# Autodesk Inventor assembly: Assembly1
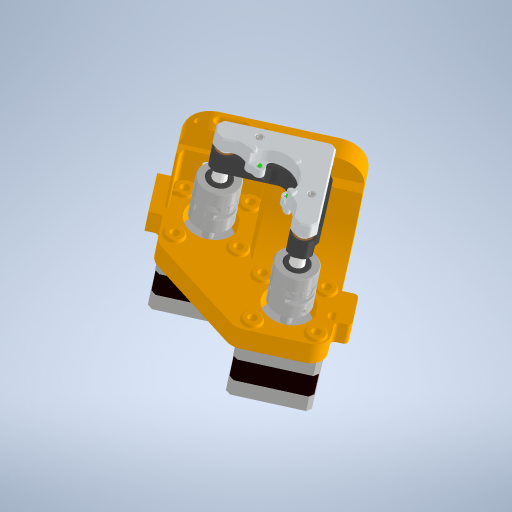
[picture p0: Inventor's stored thumbnail of the model, 512x512]
Saved by Autodesk Inventor 2024 (Build 280153000, 153)
## iProperties
Created: 2022-02-09
Part Number: Assembly1
Document SubType Name: Assembly
Designer: la8011
Author: la8011
## Documents named in this file (7)
- C:\Users\Mohamed Shehata\Dropbox (Dropbox @RU)\Design_mirror_control\Parts_assembly_final_GH\Motor_mirror_mount.iam
- C:\Users\Mohamed Shehata\Dropbox (Dropbox @RU)\Design_mirror_control\Parts_assembly_final_GH\Parts\KM1CE-Step.ipt
- C:\Users\Mohamed Shehata\Dropbox (Dropbox @RU)\Design_mirror_control\Parts_assembly_final_GH\Parts\Stage.ipt
- C:\Users\Mohamed Shehata\Dropbox (Dropbox @RU)\Design_mirror_control\Parts_assembly_final_GH\Parts\stepper.ipt
- C:\Users\Mohamed Shehata\Dropbox (Dropbox @RU)\Scan_DMD\Parts\59985K14_High-Parallel-Misalignment Flexible Shaft Coupling\59985K14_High-Parallel-Misalignment Flexible Shaft Coupling.ipt
- C:\Users\Mohamed Shehata\Dropbox (Dropbox @RU)\Scan_DMD\Parts\59985K62_93 in.-lbs. Acetal Disc for 3 4 OD High-Parallel-Misalignment Flexible Shaft Coupling\59985K62_93 in.-lbs. Acetal Disc for 3 4 OD High-Para.ipt
- C:\Users\Mohamed Shehata\Dropbox (Dropbox @RU)\Scan_DMD\Parts\59985K202_High-Parallel-Misalignment Flexible Shaft Coupling\59985K202_High-Parallel-Misalignment Flexible Shaft Coupling.ipt
## Components (10 placed, 6 different names)
1. KM1CE-Step:1 — Insert:1, Angle:3, Mate:7, Mate:14, Mate:15
2. Stage:1 — Insert:1, Angle:1, Angle:2, Angle:3, Mate:8, Mate:10, Mate:11
3. stepper:1 — Angle:1, Mate:7, Mate:8, Mate:13, Angle:6, Angle:7
4. stepper:2 — Angle:2, Mate:10, Mate:11, Mate:12, Angle:4, Angle:5
5. 59985K14_High-Parallel-Misalignment Flexible Shaft Coupling:1 — Angle:7, Mate:15, Mate:20, Mate:23
6. 59985K62_93 in.-lbs. Acetal Disc for 3 4 OD High-Para:1 — Mate:20, Mate:21, Mate:22, Mate:23
7. 59985K202_High-Parallel-Misalignment Flexible Shaft Coupling:1 — Mate:13, Angle:6, Mate:21, Mate:22
8. 59985K14_High-Parallel-Misalignment Flexible Shaft Coupling:2 — Mate:14, Angle:5, Mate:17, Mate:19
9. 59985K62_93 in.-lbs. Acetal Disc for 3 4 OD High-Para:2 — Mate:16, Mate:17, Mate:18, Mate:19
10. 59985K202_High-Parallel-Misalignment Flexible Shaft Coupling:2 — Mate:12, Angle:4, Mate:16, Mate:18
## Relationships (24: Mate 16, Angle 7, Insert 1)
- Insert:1: KM1CE-Step:1 ↔ Stage:1
- Angle:1 (0 deg): Stage:1 ↔ stepper:1
- Angle:2 (0 deg): Stage:1 ↔ stepper:2
- Angle:3 (-90 deg): KM1CE-Step:1 ↔ Stage:1
- Mate:7: KM1CE-Step:1 ↔ stepper:1
- Mate:8: Stage:1 ↔ stepper:1
- Mate:10: Stage:1 ↔ stepper:2
- Mate:11: Stage:1 ↔ stepper:2
- Mate:12: stepper:2 ↔ 59985K202_High-Parallel-Misalignment Flexible Shaft Coupling:2
- Mate:13: stepper:1 ↔ 59985K202_High-Parallel-Misalignment Flexible Shaft Coupling:1
- Mate:14: KM1CE-Step:1 ↔ 59985K14_High-Parallel-Misalignment Flexible Shaft Coupling:2
- Angle:4 (180 deg): stepper:2 ↔ 59985K202_High-Parallel-Misalignment Flexible Shaft Coupling:2
- Angle:5 (0 deg): stepper:2 ↔ 59985K14_High-Parallel-Misalignment Flexible Shaft Coupling:2
- Angle:6 (180 deg): stepper:1 ↔ 59985K202_High-Parallel-Misalignment Flexible Shaft Coupling:1
- Angle:7 (0 deg): stepper:1 ↔ 59985K14_High-Parallel-Misalignment Flexible Shaft Coupling:1
- Mate:15: KM1CE-Step:1 ↔ 59985K14_High-Parallel-Misalignment Flexible Shaft Coupling:1
- Mate:16: 59985K62_93 in.-lbs. Acetal Disc for 3 4 OD High-Para:2 ↔ 59985K202_High-Parallel-Misalignment Flexible Shaft Coupling:2
- Mate:17: 59985K14_High-Parallel-Misalignment Flexible Shaft Coupling:2 ↔ 59985K62_93 in.-lbs. Acetal Disc for 3 4 OD High-Para:2
- Mate:18: 59985K62_93 in.-lbs. Acetal Disc for 3 4 OD High-Para:2 ↔ 59985K202_High-Parallel-Misalignment Flexible Shaft Coupling:2
- Mate:19: 59985K14_High-Parallel-Misalignment Flexible Shaft Coupling:2 ↔ 59985K62_93 in.-lbs. Acetal Disc for 3 4 OD High-Para:2
- Mate:20: 59985K14_High-Parallel-Misalignment Flexible Shaft Coupling:1 ↔ 59985K62_93 in.-lbs. Acetal Disc for 3 4 OD High-Para:1
- Mate:21: 59985K62_93 in.-lbs. Acetal Disc for 3 4 OD High-Para:1 ↔ 59985K202_High-Parallel-Misalignment Flexible Shaft Coupling:1
- Mate:22: 59985K62_93 in.-lbs. Acetal Disc for 3 4 OD High-Para:1 ↔ 59985K202_High-Parallel-Misalignment Flexible Shaft Coupling:1
- Mate:23: 59985K14_High-Parallel-Misalignment Flexible Shaft Coupling:1 ↔ 59985K62_93 in.-lbs. Acetal Disc for 3 4 OD High-Para:1
